# Autodesk Inventor assembly: Body
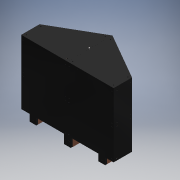
[picture p0: Inventor's stored thumbnail of the model, 180x180]
Saved by Autodesk Inventor 2017 (Build 210142000, 142)
## iProperties
Created: 2018-10-18
Part Number: Body
Document SubType Name: Assembly
Designer: Dell
Author: Dell
## Documents named in this file (5)
- C:\Users\Dell\Documents\GitHub\tr2\Body\Body.iam
- C:\Users\Dell\Documents\GitHub\tr2\Body\Body Cover Assembly.iam
- C:\Users\Dell\Documents\GitHub\tr2\Body\Body Chassis Assembly.iam
- C:\Users\Dell\Documents\GitHub\tr2\Body\BO12.ipt
- C:\Users\Dell\Documents\GitHub\tr2\Base\37d-gearmotor-50-70-encoder.ipt
## Components (4 placed, 4 different names)
1. Body Cover Assembly:1 [sub-assembly]
2. Body Chassis Assembly:1 [sub-assembly] — Mate:54, Mate:55, Flush:1, Mate:59, Mate:60, Mate:61, Mate:62
3. BO12:1 — Mate:54, Mate:55, Flush:1, Mate:56, Mate:57, Mate:58
4. 37d-gearmotor-50-70-encoder:1 — Mate:56, Mate:57, Mate:58
## Relationships (19: Mate 18, Flush 1)
- [Mate]: Body Cover Assembly:1 ↔ Body Chassis Assembly:1
- [Mate]: Body Cover Assembly:1 ↔ Body Chassis Assembly:1
- [Mate]: Body Cover Assembly:1 ↔ Body Chassis Assembly:1
- [Mate]: Body Cover Assembly:1 ↔ Body Chassis Assembly:1
- [Mate]: Body Cover Assembly:1 ↔ Body Chassis Assembly:1
- [Mate]: Body Cover Assembly:1 ↔ Body Chassis Assembly:1
- [Mate]: Body Cover Assembly:1 ↔ Body Chassis Assembly:1
- [Mate]: Body Cover Assembly:1 ↔ Body Chassis Assembly:1
- [Mate]: Body Cover Assembly:1 ↔ Body Chassis Assembly:1
- Mate:54: Body Chassis Assembly:1 ↔ BO12:1
- Mate:55: Body Chassis Assembly:1 ↔ BO12:1
- Flush:1: Body Chassis Assembly:1 ↔ BO12:1
- Mate:56: BO12:1 ↔ 37d-gearmotor-50-70-encoder:1
- Mate:57: BO12:1 ↔ 37d-gearmotor-50-70-encoder:1
- Mate:58: BO12:1 ↔ 37d-gearmotor-50-70-encoder:1
- Mate:59: Body Chassis Assembly:1
- Mate:60: Body Chassis Assembly:1
- Mate:61: Body Chassis Assembly:1
- Mate:62: Body Chassis Assembly:1
